# Autodesk Inventor assembly: Vane
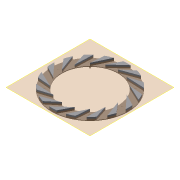
[picture p0: Inventor's stored thumbnail of the model, 180x180]
Saved by Autodesk Inventor 2022 (Build 260148000, 148)
## iProperties
Created: 2005-10-19
Part Number: Vane
Document SubType Name: Assembly
Designer: landrews
Author: landrews
## Documents named in this file (4)
- C:\Autodesk Inventor 2022 Advanced Assembly Modeling Practice Files\Mirror and Pattern\Vane.iam
- C:\Autodesk Inventor 2022 Advanced Assembly Modeling Practice Files\Mirror and Pattern\Vane_Plate.ipt
- C:\Autodesk Inventor 2022 Advanced Assembly Modeling Practice Files\Mirror and Pattern\Vane_blade.ipt
- C:\Autodesk Inventor 2022 Advanced Assembly Modeling Practice Files\Mirror and Pattern\Vane_Stud.ipt
## Components (25 placed, 3 different names)
1. Vane_Plate:1 — Mate:1, Insert:1, Flush:1, Insert:2
2. Vane_blade:1 — Mate:1, Insert:1, Angle:1
3. Vane_blade:2
4. Vane_blade:3
5. Vane_blade:4
6. Vane_blade:5
7. Vane_blade:6
8. Vane_blade:7
9. Vane_blade:8
10. Vane_blade:9
11. Vane_blade:10
12. Vane_blade:11
13. Vane_blade:12
14. Vane_blade:13
15. Vane_blade:14
16. Vane_blade:15
17. Vane_blade:16
18. Vane_Stud:1 — Insert:2
19. Vane_Stud:16
20. Vane_Stud:17
21. Vane_Stud:18
22. Vane_Stud:19
23. Vane_Stud:20
24. Vane_Stud:21
25. Vane_Stud:22
## Component patterns: (16 elements, first: Vane_blade:1), (8 elements, first: Vane_Stud:1)
## Relationships (5: Insert 2, Mate 1, Angle 1, Flush 1)
- Mate:1: Vane_Plate:1 ↔ Vane_blade:1
- Insert:1: Vane_Plate:1 ↔ Vane_blade:1
- Angle:1 (0 deg): Vane_blade:1
- Flush:1 (4.5085 mm): Vane_Plate:1
- Insert:2: Vane_Plate:1 ↔ Vane_Stud:1
